# Autodesk Inventor assembly: ASY Мешалка
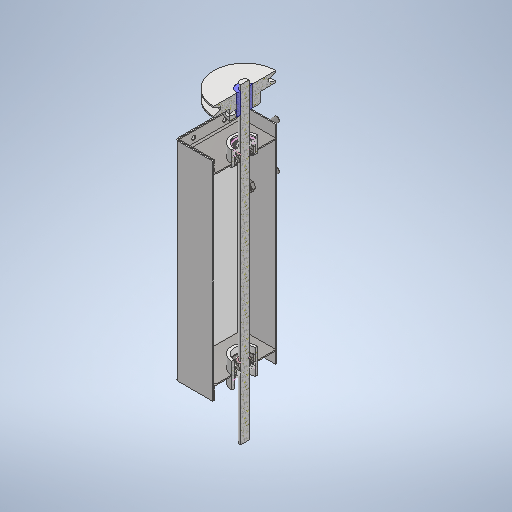
[picture p0: Inventor's stored thumbnail of the model, 512x512]
Saved by Autodesk Inventor 2025 (Build 290162010, 162A)
## iProperties
Created: 2024-04-09
Part Number: ASY Мешалка
Document SubType Name: Assembly
Designer: pokla
Author: pokla
## Documents named in this file (12)
- C:\Users\pokla\Documents\Inventor\Gusev_Meshalka\ASY Мешалка.iam
- C:\Users\pokla\Documents\Inventor\Gusev_Meshalka\SKF B7203 BE.ipt
- C:\Users\pokla\Documents\Inventor\Gusev_Meshalka\Вал.ipt
- C:\Users\pokla\Documents\Inventor\Gusev_Meshalka\CSN 02 9401 - G 17x40x7 - NBR.ipt
- C:\Users\pokla\Documents\Inventor\Gusev_Meshalka\Шкив 119 мм.ipt
- Шкив 119 мм.ipt
- C:\Users\pokla\Documents\Inventor\Gusev_Meshalka\Втулка для шкива.ipt
- C:\Users\pokla\Documents\Inventor\Content Center Files\R2024\en-US\ANSI B 27.7M(2)\ANSI B 27.7M - 3AMI-17.ipt
- C:\Users\pokla\Documents\Inventor\Content Center Files\R2024\en-US\ANSI B 27.7M(1)\ANSI B 27.7M - 3BMI-40.ipt
- C:\Users\pokla\Documents\Inventor\Gusev_Meshalka\ASY Мешалка 2.0.iam
- C:\Users\pokla\Documents\Inventor\Gusev_Meshalka\Седло для сальника.ipt
- C:\Users\pokla\Documents\Inventor\Gusev_Meshalka\Седло для подшипника.ipt
## Components (15 placed, 10 different names)
1. Вал:1 — Insert:10, Mate:13, Rigid:10, Rigid:11
2. SKF B- Angular contact SKF B7203 BE:2 — Rigid:3
3. SKF B- Angular contact SKF B7203 BE:3 — Rigid:6
4. CSN 02 9401 G G 17x40x7 - NBR:1 — Rigid:12
5. CSN 02 9401 G G 17x40x7 - NBR:2 — Rigid:13
6. Шкив 119 мм:1 — Insert:8, Mate:13
7. Втулка для шкива:1 — Insert:8, Insert:10, Rotational:1
8. ANSI B 27.7M 3AMI-17:1 — Rigid:11
9. ANSI B 27.7M 3BMI-40:1 — Rigid:7
10. ANSI B 27.7M 3BMI-40:2 — Rigid:2
11. ASY Мешалка 2.0:1 [sub-assembly] — Flush:1, Flush:2, Flush:3, Rigid:4, Rigid:5
12. Седло для сальника:2 — Rigid:4, Rigid:6, Rigid:7, Rigid:9, Rotational:1, Rigid:12
13. Седло для подшипника:1 — Rigid:2, Rigid:3, Rigid:5, Rigid:13
14. ANSI B 27.7M 3BMI-40:3 — Rigid:9
15. ANSI B 27.7M 3AMI-17:2 — Rigid:10
## Relationships (18: WeldJoint 11, Flush 3, Insert 2, Mate 1, RevoluteJoint 1)
- Insert:8: Шкив 119 мм:1 ↔ Втулка для шкива:1
- Insert:10 (10 mm): Вал:1 ↔ Втулка для шкива:1
- Mate:13: Вал:1 ↔ Шкив 119 мм:1
- Flush:1: ASY Мешалка 2.0:1
- Flush:2: ASY Мешалка 2.0:1
- Flush:3: ASY Мешалка 2.0:1
- Rigid:2 [WeldJoint]: ANSI B 27.7M 3BMI-40:2 ↔ Седло для подшипника:1
- Rigid:3 [WeldJoint]: SKF B- Angular contact SKF B7203 BE:2 ↔ Седло для подшипника:1
- Rigid:4 [WeldJoint] (23 mm): ASY Мешалка 2.0:1 ↔ Седло для сальника:2
- Rigid:5 [WeldJoint] (23 mm): ASY Мешалка 2.0:1 ↔ Седло для подшипника:1
- Rigid:6 [WeldJoint]: SKF B- Angular contact SKF B7203 BE:3 ↔ Седло для сальника:2
- Rigid:7 [WeldJoint]: ANSI B 27.7M 3BMI-40:1 ↔ Седло для сальника:2
- Rigid:9 [WeldJoint]: Седло для сальника:2 ↔ ANSI B 27.7M 3BMI-40:3
- Rotational:1 [RevoluteJoint] (50 mm): Втулка для шкива:1 ↔ Седло для сальника:2
- Rigid:10 [WeldJoint]: Вал:1 ↔ ANSI B 27.7M 3AMI-17:2
- Rigid:11 [WeldJoint]: Вал:1 ↔ ANSI B 27.7M 3AMI-17:1
- Rigid:12 [WeldJoint]: CSN 02 9401 G G 17x40x7 - NBR:1 ↔ Седло для сальника:2
- Rigid:13 [WeldJoint]: CSN 02 9401 G G 17x40x7 - NBR:2 ↔ Седло для подшипника:1
